# Autodesk Inventor assembly: tower 3
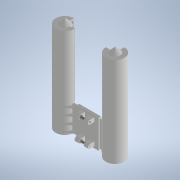
[picture p0: Inventor's stored thumbnail of the model, 180x180]
Saved by Autodesk Inventor 2020.1 (Build 241239000, 239)
## iProperties
Created: 2022-04-02
Part Number: tower 3
Document SubType Name: Assembly
Designer: User
Author: User
## Documents named in this file (6)
- D:\GitHub\TANK\3D-turret\tower 3.iam
- D:\GitHub\TANK\3D-turret\gun 3.iam
- D:\GitHub\TANK\3D-turret\gun 3_ЗЕРКАЛО1.iam
- D:\GitHub\TANK\3D-turret\верхняя защелка башни.ipt
- D:\GitHub\TANK\3D-turret\нижняя защелка пушки 2.ipt
- D:\GitHub\TANK\3D-turret\ось крепление пушки.ipt
## Components (6 placed, 5 different names)
1. gun 3:1 [sub-assembly] — Жесткий:1
2. gun 3_ЗЕРКАЛО1:1 [sub-assembly] — Жесткий:1, Жесткий:2, Жесткий:3
3. верхняя защелка башни:1 — Жесткий:2
4. нижняя защелка пушки 2:1 — Жесткий:3, Жесткий:4, Жесткий:5
5. ось крепление пушки:1 — Жесткий:5
6. ось крепление пушки:2 — Жесткий:4
## Relationships (5: WeldJoint 5)
- Жесткий:1 [WeldJoint]: gun 3:1 ↔ gun 3_ЗЕРКАЛО1:1
- Жесткий:2 [WeldJoint]: gun 3_ЗЕРКАЛО1:1 ↔ верхняя защелка башни:1
- Жесткий:3 [WeldJoint]: gun 3_ЗЕРКАЛО1:1 ↔ нижняя защелка пушки 2:1
- Жесткий:4 [WeldJoint]: нижняя защелка пушки 2:1 ↔ ось крепление пушки:2
- Жесткий:5 [WeldJoint]: нижняя защелка пушки 2:1 ↔ ось крепление пушки:1
